# Autodesk Inventor assembly: TankFlipperAssembledDriveShaft
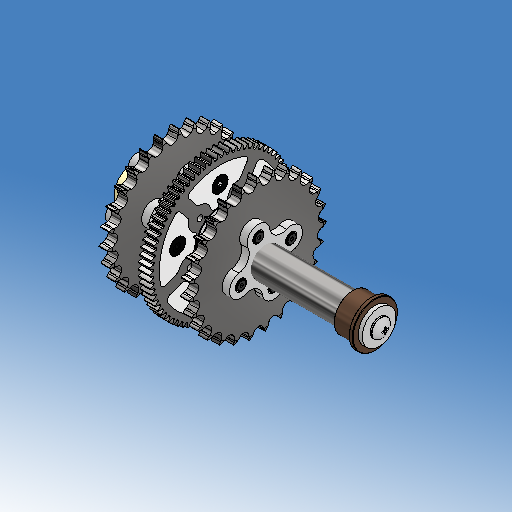
[picture p0: Inventor's stored thumbnail of the model, 512x512]
Saved by Autodesk Inventor 2025 (Build 290162000, 162)
## iProperties
Created: 2024-02-13
Part Number: TankFlipperAssembledDriveShaft
Document SubType Name: Assembly
Designer: seene
Author: seene
## Documents named in this file (17)
- C:\Users\seene\Desktop\Stony Brook\SBRT\RCR_Dexter\Drive\v1\TANK flipper\TankFlipperAssembledDriveShaft.iam
- C:\Users\seene\Desktop\Stony Brook\SBRT\RCR_Dexter\Drive\v1\TANK flipper\Drive Shaft.ipt
- C:\Users\seene\Desktop\Stony Brook\SBRT\RCR_Dexter\Drive\v1\TANK flipper\98585A121_Heavy Duty External Retaining Ring v2.ipt
- C:\Users\seene\Desktop\Stony Brook\SBRT\RCR_Dexter\Drive\v1\TANK flipper\2868T199_High-Load Oil-Embedded 863 Sleeve Bearing (1) v2(Mirror).ipt
- C:\Users\seene\Desktop\Stony Brook\SBRT\RCR_Dexter\Drive\v1\TANK flipper\Spur Gear (74 teeth).ipt
- C:\Users\seene\Desktop\Stony Brook\SBRT\RCR_Dexter\Drive\v1\TANK flipper\panel_flange.ipt
- C:\Users\seene\Desktop\Stony Brook\SBRT\RCR_Dexter\Drive\v1\TANK flipper\.25-20_FHCS_91263A553.ipt
- C:\Users\seene\Desktop\Stony Brook\SBRT\RCR_Dexter\Drive\v1\TANK flipper\bushing_2868T199.ipt
- C:\Users\seene\Desktop\Stony Brook\SBRT\RCR_Dexter\Drive\v1\TANK flipper\FlipperSpurGearMount.ipt
- C:\Users\seene\Desktop\Stony Brook\SBRT\RCR_Dexter\Drive\v1\TANK flipper\27t track drive sprocket v25.iam
- C:\Users\seene\Desktop\Stony Brook\SBRT\RCR_Dexter\Drive\v1\FlipperDriveShaft_HDPEspacer.ipt
- C:\Users\seene\Desktop\Stony Brook\SBRT\RCR_Dexter\Drive\v1\5906K523_Oil-Embedded Thrust Bronze Bearing.ipt
- C:\Users\seene\Desktop\Stony Brook\SBRT\RCR_Dexter\Drive\v1\2938T25_High-Load Oil-Embedded Sleeve Bearing.ipt
- C:\Users\seene\Desktop\Stony Brook\SBRT\RCR_Dexter\Drive\v1\FlipperDriveShaftCap.ipt
- C:\Users\seene\Desktop\Stony Brook\SBRT\RCR_Dexter\Drive\v1\90272A583_Zinc-Plated Steel Pan Head Phillips Screw_MIR.ipt
- C:\Users\seene\Desktop\Stony Brook\SBRT\RCR_Dexter\Drive\v1\98370A033_18-8 Stainless Steel Washer.ipt
- C:\Users\seene\Desktop\Stony Brook\SBRT\RCR_Dexter\Drive\v1\97063A116_1008-1010 Carbon Steel Wide-Rim Ring Shim.ipt
## Components (27 placed, 16 different names)
1. Drive Shaft:1 — Rigid:2, Rigid:3, Rigid:5, Rigid:17, Mate:9, Mate:17, Mate:19, Mate:21, Mate:22, Mate:25, Mate:27, Flush:3, Mate:28, Mate:29, Mate:34
2. 2868T199_High-Load Oil-Embedded 863 Sleeve Bearing (1) v2(Mirror):1 — Rigid:2, Rigid:18
3. 98585A121_Heavy Duty External Retaining Ring v2:2 — Rigid:3
4. 98585A121_Heavy Duty External Retaining Ring v2:3 — Rigid:5
5. Spur Gear (74 teeth):1 — Mate:1, Mate:6, Mate:7, Mate:8, Mate:9, Mate:20, Mate:37
6. panel_flange:1 — Rigid:18, Mate:23
7. panel_flange:2 — Rigid:25, Mate:16, Mate:18
8. bushing_2868T199:1 — Rigid:26, Mate:1, Flush:2
9. bushing_2868T199:2 — Rigid:26, Mate:36
10. bushing_2868T199:3 — Rigid:17, Rigid:25
11. FlipperSpurGearMount:1 — Mate:6, Mate:7, Mate:8, Mate:10, Mate:11, Mate:16, Flush:2
12. 27t track drive sprocket v25:1 [sub-assembly] — Mate:17, Mate:18, Mate:24
13. 27t track drive sprocket v25:2 [sub-assembly] — Mate:19, Mate:20, Mate:26
14. FlipperDriveShaft_HDPEspacer:1 — Mate:21, Mate:23
15. FlipperDriveShaft_HDPEspacer:2 — Mate:22, Mate:24
16. 5906K523_Oil-Embedded Thrust Bronze Bearing:1 — Mate:25, Mate:26
17. 2938T25_High-Load Oil-Embedded Sleeve Bearing:1 — Mate:27, Flush:3, Mate:35
18. FlipperDriveShaftCap:1 — Mate:28, Mate:29, Mate:30, Mate:31
19. 90272A583_Zinc-Plated Steel Pan Head Phillips Screw_MIR:1 — Mate:30, Mate:31
20. 90272A583_Zinc-Plated Steel Pan Head Phillips Screw_MIR:2 — Mate:32, Mate:33, Mate:34
21. 98370A033_18-8 Stainless Steel Washer:1 — Mate:32, Mate:33, Mate:35
22. 97063A116_1008-1010 Carbon Steel Wide-Rim Ring Shim:1 — Mate:36, Mate:37
23. .25-20_FHCS_91263A553:1 — Mate:10, Mate:11
24. .25-20_FHCS_91263A553:2
25. .25-20_FHCS_91263A553:3
26. .25-20_FHCS_91263A553:4
27. .25-20_FHCS_91263A553:5
## Component patterns: (5 elements, first: .25-20_FHCS_91263A553:1)
## Relationships (38: Mate 29, WeldJoint 7, Flush 2)
- Rigid:2 [WeldJoint]: Drive Shaft:1 ↔ 2868T199_High-Load Oil-Embedded 863 Sleeve Bearing (1) v2(Mirror):1
- Rigid:3 [WeldJoint]: Drive Shaft:1 ↔ 98585A121_Heavy Duty External Retaining Ring v2:2
- Rigid:5 [WeldJoint]: Drive Shaft:1 ↔ 98585A121_Heavy Duty External Retaining Ring v2:3
- Mate:1: Spur Gear (74 teeth):1 ↔ bushing_2868T199:1
- Rigid:17 [WeldJoint]: Drive Shaft:1 ↔ bushing_2868T199:3
- Rigid:18 [WeldJoint]: 2868T199_High-Load Oil-Embedded 863 Sleeve Bearing (1) v2(Mirror):1 ↔ panel_flange:1
- Rigid:25 [WeldJoint]: panel_flange:2 ↔ bushing_2868T199:3
- Rigid:26 [WeldJoint]: bushing_2868T199:1 ↔ bushing_2868T199:2
- Mate:6: Spur Gear (74 teeth):1 ↔ FlipperSpurGearMount:1
- Mate:7: Spur Gear (74 teeth):1 ↔ FlipperSpurGearMount:1
- Mate:8: Spur Gear (74 teeth):1 ↔ FlipperSpurGearMount:1
- Mate:9: Drive Shaft:1 ↔ Spur Gear (74 teeth):1
- Mate:10: FlipperSpurGearMount:1 ↔ .25-20_FHCS_91263A553:1
- Mate:11: FlipperSpurGearMount:1 ↔ .25-20_FHCS_91263A553:1
- Mate:16 (6.35 mm): panel_flange:2 ↔ FlipperSpurGearMount:1
- Flush:2: bushing_2868T199:1 ↔ FlipperSpurGearMount:1
- Mate:17: Drive Shaft:1 ↔ 27t track drive sprocket v25:1
- Mate:18 (5.0932 mm): panel_flange:2 ↔ 27t track drive sprocket v25:1
- Mate:19: Drive Shaft:1 ↔ 27t track drive sprocket v25:2
- Mate:20 (23.8125 mm): Spur Gear (74 teeth):1 ↔ 27t track drive sprocket v25:2
- Mate:21: Drive Shaft:1 ↔ FlipperDriveShaft_HDPEspacer:1
- Mate:22: Drive Shaft:1 ↔ FlipperDriveShaft_HDPEspacer:2
- Mate:23: panel_flange:1 ↔ FlipperDriveShaft_HDPEspacer:1
- Mate:24: 27t track drive sprocket v25:1 ↔ FlipperDriveShaft_HDPEspacer:2
- Mate:25: Drive Shaft:1 ↔ 5906K523_Oil-Embedded Thrust Bronze Bearing:1
- Mate:26: 27t track drive sprocket v25:2 ↔ 5906K523_Oil-Embedded Thrust Bronze Bearing:1
- Mate:27: Drive Shaft:1 ↔ 2938T25_High-Load Oil-Embedded Sleeve Bearing:1
- Flush:3: Drive Shaft:1 ↔ 2938T25_High-Load Oil-Embedded Sleeve Bearing:1
- Mate:28: Drive Shaft:1 ↔ FlipperDriveShaftCap:1
- Mate:29: Drive Shaft:1 ↔ FlipperDriveShaftCap:1
- Mate:30: FlipperDriveShaftCap:1 ↔ 90272A583_Zinc-Plated Steel Pan Head Phillips Screw_MIR:1
- Mate:31: FlipperDriveShaftCap:1 ↔ 90272A583_Zinc-Plated Steel Pan Head Phillips Screw_MIR:1
- Mate:32: 90272A583_Zinc-Plated Steel Pan Head Phillips Screw_MIR:2 ↔ 98370A033_18-8 Stainless Steel Washer:1
- Mate:33: 90272A583_Zinc-Plated Steel Pan Head Phillips Screw_MIR:2 ↔ 98370A033_18-8 Stainless Steel Washer:1
- Mate:34: Drive Shaft:1 ↔ 90272A583_Zinc-Plated Steel Pan Head Phillips Screw_MIR:2
- Mate:35: 2938T25_High-Load Oil-Embedded Sleeve Bearing:1 ↔ 98370A033_18-8 Stainless Steel Washer:1
- Mate:36: bushing_2868T199:2 ↔ 97063A116_1008-1010 Carbon Steel Wide-Rim Ring Shim:1
- Mate:37: Spur Gear (74 teeth):1 ↔ 97063A116_1008-1010 Carbon Steel Wide-Rim Ring Shim:1
